# Autodesk Inventor assembly: outer_mirrored
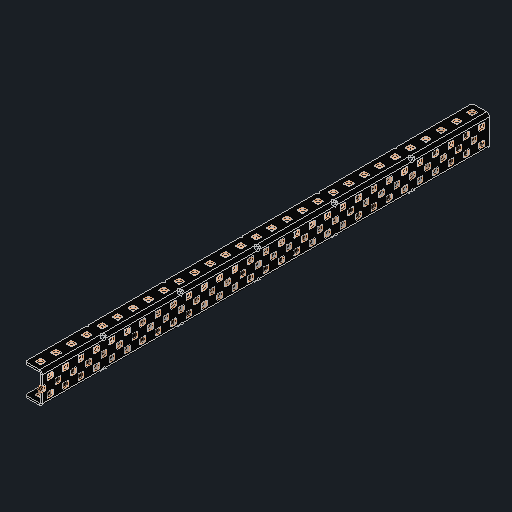
[picture p0: Inventor's stored thumbnail of the model, 512x512]
Saved by Autodesk Inventor 2024 (Build 280153000, 153)
## iProperties
Created: 2024-05-12
Part Number: outer_mirrored
Document SubType Name: Assembly
Designer: Averey Ku
Author: Averey Ku
## Documents named in this file (4)
- D:\vex_robotics\hardware\cad\kdot\chassis\drivebay\mirrored_parts\outer_mirrored.iam
- D:\vex_robotics\hardware\cad\kdot\chassis\drivebay\mirrored_parts\Alu C 1x2x1x29_mirrored.ipt
- D:\vex_robotics\hardware\cad\kdot\chassis\drivebay\mirrored_parts\Bearing Flat Low Profile_mirrored.ipt
- D:\vex_robotics\hardware\cad\kdot\chassis\drivebay\mirrored_parts\.375 OD Aluminum Spacer 0.875_mirrored.ipt
## Components (10 placed, 3 different names)
1. Alu C 1x2x1x29_mirrored:1 — Mate:8, Insert:8, Mate:2, Insert:2, Mate:3, Insert:3, Mate:4, Insert:4, Mate:5, Insert:5, Mate:6, Insert:6, Mate:7, Insert:7, Insert:10, Insert:9
2. Bearing Flat Low Profile_mirrored:1 — Mate:8, Insert:8
3. Bearing Flat Low Profile_mirrored:2 — Mate:2, Insert:2
4. Bearing Flat Low Profile_mirrored:3 — Mate:3, Insert:3
5. Bearing Flat Low Profile_mirrored:4 — Mate:4, Insert:4
6. Bearing Flat Low Profile_mirrored:5 — Mate:5, Insert:5
7. Bearing Flat Low Profile_mirrored:6 — Mate:6, Insert:6
8. Bearing Flat Low Profile_mirrored:7 — Mate:7, Insert:7
9. .375 OD Aluminum Spacer 0.875_mirrored:1 — Insert:10
10. .375 OD Aluminum Spacer 0.875_mirrored:2 — Insert:9
## Relationships (16: Insert 9, Mate 7)
- Mate:8: Alu C 1x2x1x29_mirrored:1 ↔ Bearing Flat Low Profile_mirrored:1
- Insert:8: Alu C 1x2x1x29_mirrored:1 ↔ Bearing Flat Low Profile_mirrored:1
- Mate:2: Alu C 1x2x1x29_mirrored:1 ↔ Bearing Flat Low Profile_mirrored:2
- Insert:2: Alu C 1x2x1x29_mirrored:1 ↔ Bearing Flat Low Profile_mirrored:2
- Mate:3: Alu C 1x2x1x29_mirrored:1 ↔ Bearing Flat Low Profile_mirrored:3
- Insert:3: Alu C 1x2x1x29_mirrored:1 ↔ Bearing Flat Low Profile_mirrored:3
- Mate:4: Alu C 1x2x1x29_mirrored:1 ↔ Bearing Flat Low Profile_mirrored:4
- Insert:4: Alu C 1x2x1x29_mirrored:1 ↔ Bearing Flat Low Profile_mirrored:4
- Mate:5: Alu C 1x2x1x29_mirrored:1 ↔ Bearing Flat Low Profile_mirrored:5
- Insert:5: Alu C 1x2x1x29_mirrored:1 ↔ Bearing Flat Low Profile_mirrored:5
- Mate:6: Alu C 1x2x1x29_mirrored:1 ↔ Bearing Flat Low Profile_mirrored:6
- Insert:6: Alu C 1x2x1x29_mirrored:1 ↔ Bearing Flat Low Profile_mirrored:6
- Mate:7: Alu C 1x2x1x29_mirrored:1 ↔ Bearing Flat Low Profile_mirrored:7
- Insert:7: Alu C 1x2x1x29_mirrored:1 ↔ Bearing Flat Low Profile_mirrored:7
- Insert:10: Alu C 1x2x1x29_mirrored:1 ↔ .375 OD Aluminum Spacer 0.875_mirrored:1
- Insert:9: Alu C 1x2x1x29_mirrored:1 ↔ .375 OD Aluminum Spacer 0.875_mirrored:2
